# Autodesk Inventor assembly: light_holder
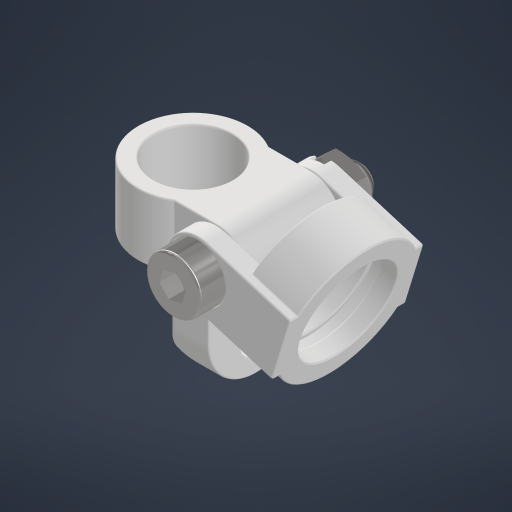
[picture p0: Inventor's stored thumbnail of the model, 512x512]
Saved by Autodesk Inventor 2023 (Build 270158000, 158)
## iProperties
Created: 2022-05-28
Part Number: light_holder
Document SubType Name: Assembly
Designer: Norbert Ligas
Author: Norbert Ligas
## Documents named in this file (5)
- C:\Users\norbe\Repozytoria\NormalMapScanner\stand_construction\parts\light_holder.iam
- C:\Users\norbe\Repozytoria\NormalMapScanner\stand_construction\parts\light_holder_part1.ipt
- C:\Users\norbe\Repozytoria\NormalMapScanner\stand_construction\parts\light_holder_part2.ipt
- C:\Users\norbe\OneDrive\Dokumenty\Inventor\Content Center Files\R2023\en-US\ISO 4762(2)\ISO 4762 - M4 x 20ISO.ipt
- C:\Users\norbe\OneDrive\Dokumenty\Inventor\Content Center Files\R2023\en-US\ISO 4032(2)\ISO 4032 - M4 - ISO.ipt
## Components (4 placed, 4 different names)
1. light_holder_part1:1 — Rotational:1, Rotational:2, Insert:1, Mate:3, Mate:4
2. light_holder_part2:1 — Flush:1, Flush:2, Mate:1, Rotational:1, Rotational:2
3. ISO 4762 M4 x 20:1 — Insert:1, Mate:2
4. ISO 4032 M4:1 — Mate:2, Mate:3, Mate:4
## Relationships (9: Mate 4, Flush 2, RevoluteJoint 2, Insert 1)
- Flush:1: light_holder_part2:1
- Flush:2: light_holder_part2:1
- Mate:1: light_holder_part2:1
- Rotational:1 [RevoluteJoint]: light_holder_part1:1 ↔ light_holder_part2:1
- Rotational:2 [RevoluteJoint]: light_holder_part1:1 ↔ light_holder_part2:1
- Insert:1: light_holder_part1:1 ↔ ISO 4762 M4 x 20:1
- Mate:2: ISO 4762 M4 x 20:1 ↔ ISO 4032 M4:1
- Mate:3: light_holder_part1:1 ↔ ISO 4032 M4:1
- Mate:4: light_holder_part1:1 ↔ ISO 4032 M4:1
